# Autodesk Inventor assembly: rear bike light
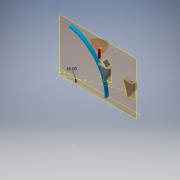
[picture p0: Inventor's stored thumbnail of the model, 180x180]
Saved by Autodesk Inventor 2016 (Build 200138000, 138)
## iProperties
Created: 2017-09-18
Part Number: rear bike light
Document SubType Name: Assembly
Designer: Student
Author: Student
## Documents named in this file (7)
- C:\Users\Student\Documents\GitHub\bikelightmount\rear bike light.iam
- C:\Users\Student\Documents\GitHub\bikelightmount\Part2.ipt
- C:\Users\Student\Documents\GitHub\bikelightmount\light.ipt
- C:\Users\Student\Documents\GitHub\bikelightmount\light_mount.ipt
- C:\Users\Student\Documents\GitHub\bikelightmount\LightMount2.ipt
- C:\Users\Student\Documents\GitHub\bikelightmount\base model.ipt
- C:\Users\Student\Documents\High_Mount.ipt
## Components (7 placed, 6 different names)
1. Part2:1 — Flush:2
2. light:1 — Flush:5
3. light_mount:1
4. LightMount2:1 — Flush:3, Flush:4
5. base model:1
6. High_Mount:1 — Flush:5
7. base model:4
## Relationships (4: Flush 4)
- Flush:2: Part2:1
- Flush:3: LightMount2:1
- Flush:4: LightMount2:1
- Flush:5: light:1 ↔ High_Mount:1
